# Autodesk Inventor assembly: ZMR250 Quadcopter Frame -Assembly
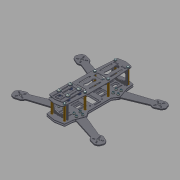
[picture p0: Inventor's stored thumbnail of the model, 180x180]
Saved by Autodesk Inventor 2011 SP2 (Build 150309200, 309)
## iProperties
Created: 2015-02-19
Part Number: ZMR250 Quadcopter Frame -Assembly
Document SubType Name: Assembly
Designer: Greg Pavlik
Author: Greg Pavlik
## Documents named in this file (15)
- C:\Users\Greg\Desktop\ZMR250 Quadcopter Frame\ZMR250 Quadcopter Frame -Assembly.iam
- C:\Users\Greg\Desktop\ZMR250 Quadcopter Frame\Bottom Plate.ipt
- C:\Users\Greg\Desktop\ZMR250 Quadcopter Frame\Arm.ipt
- C:\Users\Greg\Desktop\ZMR250 Quadcopter Frame\Spacer.ipt
- C:\Users\Greg\Desktop\ZMR250 Quadcopter Frame\Top Plate.ipt
- C:\Users\Greg\Desktop\ZMR250 Quadcopter Frame\Damper.ipt
- C:\Users\Greg\Desktop\ZMR250 Quadcopter Frame\Camera Plate.ipt
- C:\Users\Greg\Desktop\ZMR250 Quadcopter Frame\FPV Plate.ipt
- C:\Users\Greg\Desktop\ZMR250 Quadcopter Frame\Lock Washer.ipt
- C:\Users\Greg\Desktop\ZMR250 Quadcopter Frame\Hex Socket Screw.ipt
- C:\Users\Greg\Desktop\ZMR250 Quadcopter Frame\Hex Nut with Washer Face.ipt
- C:\Users\Greg\Desktop\ZMR250 Quadcopter Frame\Hex Head Cap Screw.ipt
- C:\Users\Greg\Desktop\ZMR250 Quadcopter Frame\Lock Washer -2.ipt
- C:\Users\Greg\Desktop\ZMR250 Quadcopter Frame\Round Head Machine Screw.ipt
- C:\Users\Greg\Desktop\ZMR250 Quadcopter Frame\Hex Jam Nut with Washer Face.ipt
## Components (134 placed, 14 different names)
1. Bottom Plate:1 — Flush:1, Flush:2, Mate:1, Mate:2, Mate:3, Mate:4, Mate:5, Mate:6, Mate:7, Mate:8, Mate:9, Mate:10, Mate:11, Mate:12, Mate:53, Mate:54, Insert:21, Insert:22, Insert:23, Insert:24, Insert:25, Insert:26, Insert:27, Insert:28, Insert:29, Insert:30, Insert:31, Insert:32, Insert:57, Insert:58, Insert:59, Insert:60, Insert:61, Insert:62, Insert:63, Insert:64
2. Bottom Plate:2 — Flush:1, Flush:2, Mate:13, Mate:14, Mate:15, Mate:16, Mate:17, Mate:18, Mate:19, Mate:20, Mate:21, Mate:22, Mate:23, Mate:24, Mate:25, Mate:26, Mate:27, Mate:28, Mate:29, Flush:7, Mate:41, Mate:42, Mate:43, Mate:44, Mate:45, Mate:46, Mate:47, Mate:48, Mate:49, Mate:50, Mate:51, Mate:52, Insert:9, Insert:10, Insert:11, Insert:12, Insert:13, Insert:14, Insert:15, Insert:16, Insert:17, Insert:18, Insert:19, Insert:20
3. Arm:1 — Mate:5, Mate:8, Mate:9
4. Arm:2 — Mate:6, Mate:7, Mate:12, Mate:13
5. Arm:3 — Mate:1, Mate:2, Mate:11
6. Arm:4 — Mate:3, Mate:4, Mate:10
7. Spacer:1 — Mate:15, Mate:27
8. Spacer:2 — Mate:20, Mate:29
9. Spacer:3 — Mate:21, Mate:28
10. Spacer:4 — Mate:14, Mate:22, Mate:31, Mate:32
11. Spacer:5 — Mate:16, Mate:26
12. Spacer:6 — Mate:17, Mate:23, Mate:30
13. Spacer:7 — Mate:18, Mate:24
14. Spacer:8 — Mate:19, Mate:25
15. Top Plate:1 — Mate:30, Mate:31, Mate:32, Mate:33, Mate:34, Mate:35, Mate:36, Mate:37, Insert:73, Insert:74, Insert:75, Insert:76, Insert:77, Insert:78, Insert:79, Insert:80
16. Damper:1 — Mate:33, Flush:5, Insert:92, Insert:94
17. Damper:2 — Mate:34, Flush:3, Flush:4, Mate:38, Mate:40, Insert:89, Insert:96
18. Damper:3 — Mate:35, Flush:4, Mate:37, Insert:91, Insert:95
19. Damper:4 — Mate:36, Flush:3, Flush:5, Mate:39, Insert:90, Insert:93
20. Camera Plate:1 — Mate:38, Mate:39, Mate:40
21. FPV Plate:1 — Flush:6, Flush:7, Mate:41, Mate:44
22. FPV Plate:2 — Flush:6, Mate:42, Mate:43
23. Lock Washer:1 — Flush:8, Mate:49, Insert:4
24. Lock Washer:2 — Flush:8, Flush:9, Mate:48, Insert:3
25. Lock Washer:3 — Flush:9, Flush:10, Mate:47, Insert:2
26. Lock Washer:4 — Flush:10, Mate:45, Mate:46, Insert:1
27. Lock Washer:5 — Flush:11, Mate:54, Insert:5
28. Lock Washer:6 — Mate:52, Flush:11, Flush:12, Insert:7
29. Lock Washer:7 — Mate:50, Flush:12, Flush:13, Mate:53, Insert:6
30. Lock Washer:8 — Mate:51, Flush:13, Insert:8
31. Lock Washer:9 — Insert:9, Insert:47
32. Lock Washer:10 — Insert:10, Insert:45
33. Lock Washer:11 — Insert:11, Insert:46
34. Lock Washer:12 — Insert:12, Insert:48
35. Lock Washer:13 — Insert:26, Insert:38
36. Lock Washer:14 — Insert:27, Insert:37
37. Lock Washer:15 — Insert:28, Insert:39
38. Lock Washer:16 — Insert:29, Insert:41
39. Lock Washer:17 — Insert:17, Insert:54
40. Lock Washer:18 — Insert:20, Insert:55
41. Lock Washer:19 — Insert:19, Insert:53
42. Lock Washer:20 — Insert:18, Insert:56
43. Lock Washer:21 — Insert:23, Insert:34
44. Lock Washer:22 — Insert:24, Insert:36
45. Lock Washer:23 — Insert:21, Insert:33
46. Lock Washer:24 — Insert:22, Insert:35
47. Lock Washer:25 — Insert:13, Insert:49
48. Lock Washer:26 — Insert:14, Insert:50
49. Lock Washer:27 — Insert:15, Insert:52
50. Lock Washer:28 — Insert:30, Insert:42
51. Lock Washer:29 — Insert:16, Insert:51
52. Lock Washer:30 — Insert:25, Insert:40
53. Lock Washer:31 — Insert:31, Insert:43
54. Lock Washer:32 — Insert:32, Insert:44
55. Hex Socket Screw:4 — Insert:4
56. Hex Nut with Washer Face:1 — Insert:8
57. Hex Nut with Washer Face:2 — Insert:7
58. Hex Nut with Washer Face:3 — Insert:5
59. Hex Nut with Washer Face:4 — Insert:6
60. Hex Nut with Washer Face:5 — Insert:41
61. Hex Nut with Washer Face:6 — Insert:42
62. Hex Nut with Washer Face:7 — Insert:43
63. Hex Nut with Washer Face:8 — Insert:44
64. Hex Nut with Washer Face:9 — Insert:37
65. Hex Nut with Washer Face:10 — Insert:38
66. Hex Nut with Washer Face:11 — Insert:39
67. Hex Nut with Washer Face:12 — Insert:40
68. Hex Nut with Washer Face:13 — Insert:36
69. Hex Nut with Washer Face:14 — Insert:35
70. Hex Nut with Washer Face:15 — Insert:34
71. Hex Nut with Washer Face:16 — Insert:33
72. Hex Socket Screw:1 — Insert:1
73. Hex Socket Screw:2 — Insert:2
74. Hex Socket Screw:3 — Insert:3
75. Hex Socket Screw:5 — Insert:49
76. Hex Socket Screw:6 — Insert:50
77. Hex Socket Screw:7 — Insert:51
78. Hex Socket Screw:8 — Insert:52
79. Hex Socket Screw:9 — Insert:53
80. Hex Socket Screw:10 — Insert:54
81. Hex Socket Screw:11 — Insert:55
82. Hex Socket Screw:12 — Insert:56
83. Hex Socket Screw:13 — Insert:45
84. Hex Socket Screw:14 — Insert:46
85. Hex Socket Screw:15 — Insert:47
86. Hex Socket Screw:16 — Insert:48
87. Lock Washer:33 — Insert:60, Insert:66
88. Lock Washer:34 — Insert:59, Insert:65
89. Lock Washer:35 — Insert:61, Insert:67
90. Lock Washer:36 — Insert:62, Insert:68
91. Lock Washer:37 — Insert:63, Insert:69
92. Lock Washer:38 — Insert:58, Insert:71
93. Lock Washer:39 — Insert:57, Insert:72
94. Lock Washer:40 — Insert:64, Insert:70
95. Hex Nut with Washer Face:17 — Insert:71
96. Hex Nut with Washer Face:18 — Insert:72
97. Hex Nut with Washer Face:19 — Insert:70
98. Hex Nut with Washer Face:20 — Insert:69
99. Hex Nut with Washer Face:21 — Insert:68
100. Hex Nut with Washer Face:22 — Insert:67
101. Hex Nut with Washer Face:23 — Insert:65
102. Hex Nut with Washer Face:24 — Insert:66
103. Lock Washer:41 — Insert:77, Insert:86
104. Lock Washer:42 — Insert:76, Insert:83
105. Lock Washer:43 — Insert:78, Insert:82
106. Lock Washer:44 — Insert:79, Insert:81
107. Lock Washer:45 — Insert:80, Insert:85
108. Lock Washer:46 — Insert:75, Insert:87
109. Lock Washer:47 — Insert:74, Insert:88
110. Lock Washer:48 — Insert:73, Insert:84
111. Hex Head Cap Screw:1 — Insert:81
112. Hex Head Cap Screw:2 — Insert:82
113. Hex Head Cap Screw:3 — Insert:83
114. Hex Head Cap Screw:4 — Insert:84
115. Hex Head Cap Screw:5 — Insert:85
116. Hex Head Cap Screw:6 — Insert:86
117. Hex Head Cap Screw:7 — Insert:87
118. Hex Head Cap Screw:8 — Insert:88
119. Lock Washer -2:1 — Insert:92, Insert:98
120. Lock Washer -2:2 — Insert:96, Insert:104
121. Lock Washer -2:3 — Insert:90, Insert:97
122. Lock Washer -2:4 — Insert:93, Insert:101
123. Lock Washer -2:5 — Insert:89, Insert:100
124. Lock Washer -2:6 — Insert:91, Insert:99
125. Lock Washer -2:7 — Insert:94, Insert:102
126. Lock Washer -2:8 — Insert:95, Insert:103
127. Round Head Machine Screw:1 — Insert:97
128. Round Head Machine Screw:2 — Insert:98
129. Round Head Machine Screw:3 — Insert:99
130. Round Head Machine Screw:4 — Insert:100
131. Hex Jam Nut with Washer Face:1 — Insert:101
132. Hex Jam Nut with Washer Face:2 — Insert:102
133. Hex Jam Nut with Washer Face:3 — Insert:104
134. Hex Jam Nut with Washer Face:4 — Insert:103
## Relationships (171: Insert 104, Mate 54, Flush 13)
- Flush:1: Bottom Plate:1 ↔ Bottom Plate:2
- Flush:2: Bottom Plate:1 ↔ Bottom Plate:2
- Mate:1: Bottom Plate:1 ↔ Arm:3
- Mate:2: Bottom Plate:1 ↔ Arm:3
- Mate:3: Bottom Plate:1 ↔ Arm:4
- Mate:4: Bottom Plate:1 ↔ Arm:4
- Mate:5: Bottom Plate:1 ↔ Arm:1
- Mate:6: Bottom Plate:1 ↔ Arm:2
- Mate:7: Bottom Plate:1 ↔ Arm:2
- Mate:8: Bottom Plate:1 ↔ Arm:1
- Mate:9: Bottom Plate:1 ↔ Arm:1
- Mate:10: Bottom Plate:1 ↔ Arm:4
- Mate:11: Bottom Plate:1 ↔ Arm:3
- Mate:12: Bottom Plate:1 ↔ Arm:2
- Mate:13: Bottom Plate:2 ↔ Arm:2
- Mate:14: Bottom Plate:2 ↔ Spacer:4
- Mate:15: Bottom Plate:2 ↔ Spacer:1
- Mate:16: Bottom Plate:2 ↔ Spacer:5
- Mate:17: Bottom Plate:2 ↔ Spacer:6
- Mate:18: Bottom Plate:2 ↔ Spacer:7
- Mate:19: Bottom Plate:2 ↔ Spacer:8
- Mate:20: Bottom Plate:2 ↔ Spacer:2
- Mate:21: Bottom Plate:2 ↔ Spacer:3
- Mate:22: Bottom Plate:2 ↔ Spacer:4
- Mate:23: Bottom Plate:2 ↔ Spacer:6
- Mate:24: Bottom Plate:2 ↔ Spacer:7
- Mate:25: Bottom Plate:2 ↔ Spacer:8
- Mate:26: Bottom Plate:2 ↔ Spacer:5
- Mate:27: Bottom Plate:2 ↔ Spacer:1
- Mate:28: Bottom Plate:2 ↔ Spacer:3
- Mate:29: Bottom Plate:2 ↔ Spacer:2
- Mate:30: Spacer:6 ↔ Top Plate:1
- Mate:31: Spacer:4 ↔ Top Plate:1
- Mate:32: Spacer:4 ↔ Top Plate:1
- Mate:33: Top Plate:1 ↔ Damper:1
- Mate:34: Top Plate:1 ↔ Damper:2
- Mate:35: Top Plate:1 ↔ Damper:3
- Mate:36: Top Plate:1 ↔ Damper:4
- Flush:3: Damper:2 ↔ Damper:4
- Flush:4: Damper:2 ↔ Damper:3
- Flush:5: Damper:1 ↔ Damper:4
- Mate:37: Top Plate:1 ↔ Damper:3
- Mate:38: Damper:2 ↔ Camera Plate:1
- Mate:39: Damper:4 ↔ Camera Plate:1
- Mate:40: Damper:2 ↔ Camera Plate:1
- Flush:6: FPV Plate:1 ↔ FPV Plate:2
- Flush:7: Bottom Plate:2 ↔ FPV Plate:1
- Mate:41: Bottom Plate:2 ↔ FPV Plate:1
- Mate:42: Bottom Plate:2 ↔ FPV Plate:2
- Mate:43: Bottom Plate:2 ↔ FPV Plate:2
- Mate:44: Bottom Plate:2 ↔ FPV Plate:1
- Flush:8: Lock Washer:1 ↔ Lock Washer:2
- Flush:9: Lock Washer:2 ↔ Lock Washer:3
- Flush:10: Lock Washer:3 ↔ Lock Washer:4
- Mate:45: Bottom Plate:2 ↔ Lock Washer:4
- Mate:46: Bottom Plate:2 ↔ Lock Washer:4
- Mate:47: Bottom Plate:2 ↔ Lock Washer:3
- Mate:48: Bottom Plate:2 ↔ Lock Washer:2
- Mate:49: Bottom Plate:2 ↔ Lock Washer:1
- Mate:50: Bottom Plate:2 ↔ Lock Washer:7
- Mate:51: Bottom Plate:2 ↔ Lock Washer:8
- Mate:52: Bottom Plate:2 ↔ Lock Washer:6
- Flush:11: Lock Washer:5 ↔ Lock Washer:6
- Flush:12: Lock Washer:6 ↔ Lock Washer:7
- Flush:13: Lock Washer:7 ↔ Lock Washer:8
- Mate:53: Bottom Plate:1 ↔ Lock Washer:7
- Mate:54: Bottom Plate:1 ↔ Lock Washer:5
- Insert:1: Lock Washer:4 ↔ Hex Socket Screw:1
- Insert:2: Lock Washer:3 ↔ Hex Socket Screw:2
- Insert:3: Lock Washer:2 ↔ Hex Socket Screw:3
- Insert:4: Lock Washer:1 ↔ Hex Socket Screw:4
- Insert:5: Lock Washer:5 ↔ Hex Nut with Washer Face:3
- Insert:6: Lock Washer:7 ↔ Hex Nut with Washer Face:4
- Insert:7: Lock Washer:6 ↔ Hex Nut with Washer Face:2
- Insert:8: Lock Washer:8 ↔ Hex Nut with Washer Face:1
- Insert:9: Bottom Plate:2 ↔ Lock Washer:9
- Insert:10: Bottom Plate:2 ↔ Lock Washer:10
- Insert:11: Bottom Plate:2 ↔ Lock Washer:11
- Insert:12: Bottom Plate:2 ↔ Lock Washer:12
- Insert:13: Bottom Plate:2 ↔ Lock Washer:25
- Insert:14: Bottom Plate:2 ↔ Lock Washer:26
- Insert:15: Bottom Plate:2 ↔ Lock Washer:27
- Insert:16: Bottom Plate:2 ↔ Lock Washer:29
- Insert:17: Bottom Plate:2 ↔ Lock Washer:17
- Insert:18: Bottom Plate:2 ↔ Lock Washer:20
- Insert:19: Bottom Plate:2 ↔ Lock Washer:19
- Insert:20: Bottom Plate:2 ↔ Lock Washer:18
- Insert:21: Bottom Plate:1 ↔ Lock Washer:23
- Insert:22: Bottom Plate:1 ↔ Lock Washer:24
- Insert:23: Bottom Plate:1 ↔ Lock Washer:21
- Insert:24: Bottom Plate:1 ↔ Lock Washer:22
- Insert:25: Bottom Plate:1 ↔ Lock Washer:30
- Insert:26: Bottom Plate:1 ↔ Lock Washer:13
- Insert:27: Bottom Plate:1 ↔ Lock Washer:14
- Insert:28: Bottom Plate:1 ↔ Lock Washer:15
- Insert:29: Bottom Plate:1 ↔ Lock Washer:16
- Insert:30: Bottom Plate:1 ↔ Lock Washer:28
- Insert:31: Bottom Plate:1 ↔ Lock Washer:31
- Insert:32: Bottom Plate:1 ↔ Lock Washer:32
- Insert:33: Lock Washer:23 ↔ Hex Nut with Washer Face:16
- Insert:34: Lock Washer:21 ↔ Hex Nut with Washer Face:15
- Insert:35: Lock Washer:24 ↔ Hex Nut with Washer Face:14
- Insert:36: Lock Washer:22 ↔ Hex Nut with Washer Face:13
- Insert:37: Lock Washer:14 ↔ Hex Nut with Washer Face:9
- Insert:38: Lock Washer:13 ↔ Hex Nut with Washer Face:10
- Insert:39: Lock Washer:15 ↔ Hex Nut with Washer Face:11
- Insert:40: Lock Washer:30 ↔ Hex Nut with Washer Face:12
- Insert:41: Lock Washer:16 ↔ Hex Nut with Washer Face:5
- Insert:42: Lock Washer:28 ↔ Hex Nut with Washer Face:6
- Insert:43: Lock Washer:31 ↔ Hex Nut with Washer Face:7
- Insert:44: Lock Washer:32 ↔ Hex Nut with Washer Face:8
- Insert:45: Lock Washer:10 ↔ Hex Socket Screw:13
- Insert:46: Lock Washer:11 ↔ Hex Socket Screw:14
- Insert:47: Lock Washer:9 ↔ Hex Socket Screw:15
- Insert:48: Lock Washer:12 ↔ Hex Socket Screw:16
- Insert:49: Lock Washer:25 ↔ Hex Socket Screw:5
- Insert:50: Lock Washer:26 ↔ Hex Socket Screw:6
- Insert:51: Lock Washer:29 ↔ Hex Socket Screw:7
- Insert:52: Lock Washer:27 ↔ Hex Socket Screw:8
- Insert:53: Lock Washer:19 ↔ Hex Socket Screw:9
- Insert:54: Lock Washer:17 ↔ Hex Socket Screw:10
- Insert:55: Lock Washer:18 ↔ Hex Socket Screw:11
- Insert:56: Lock Washer:20 ↔ Hex Socket Screw:12
- Insert:57: Bottom Plate:1 ↔ Lock Washer:39
- Insert:58: Bottom Plate:1 ↔ Lock Washer:38
- Insert:59: Bottom Plate:1 ↔ Lock Washer:34
- Insert:60: Bottom Plate:1 ↔ Lock Washer:33
- Insert:61: Bottom Plate:1 ↔ Lock Washer:35
- Insert:62: Bottom Plate:1 ↔ Lock Washer:36
- Insert:63: Bottom Plate:1 ↔ Lock Washer:37
- Insert:64: Bottom Plate:1 ↔ Lock Washer:40
- Insert:65: Lock Washer:34 ↔ Hex Nut with Washer Face:23
- Insert:66: Lock Washer:33 ↔ Hex Nut with Washer Face:24
- Insert:67: Lock Washer:35 ↔ Hex Nut with Washer Face:22
- Insert:68: Lock Washer:36 ↔ Hex Nut with Washer Face:21
- Insert:69: Lock Washer:37 ↔ Hex Nut with Washer Face:20
- Insert:70: Lock Washer:40 ↔ Hex Nut with Washer Face:19
- Insert:71: Lock Washer:38 ↔ Hex Nut with Washer Face:17
- Insert:72: Lock Washer:39 ↔ Hex Nut with Washer Face:18
- Insert:73: Top Plate:1 ↔ Lock Washer:48
- Insert:74: Top Plate:1 ↔ Lock Washer:47
- Insert:75: Top Plate:1 ↔ Lock Washer:46
- Insert:76: Top Plate:1 ↔ Lock Washer:42
- Insert:77: Top Plate:1 ↔ Lock Washer:41
- Insert:78: Top Plate:1 ↔ Lock Washer:43
- Insert:79: Top Plate:1 ↔ Lock Washer:44
- Insert:80: Top Plate:1 ↔ Lock Washer:45
- Insert:81: Lock Washer:44 ↔ Hex Head Cap Screw:1
- Insert:82: Lock Washer:43 ↔ Hex Head Cap Screw:2
- Insert:83: Lock Washer:42 ↔ Hex Head Cap Screw:3
- Insert:84: Lock Washer:48 ↔ Hex Head Cap Screw:4
- Insert:85: Lock Washer:45 ↔ Hex Head Cap Screw:5
- Insert:86: Lock Washer:41 ↔ Hex Head Cap Screw:6
- Insert:87: Lock Washer:46 ↔ Hex Head Cap Screw:7
- Insert:88: Lock Washer:47 ↔ Hex Head Cap Screw:8
- Insert:89: Damper:2 ↔ Lock Washer -2:5
- Insert:90: Damper:4 ↔ Lock Washer -2:3
- Insert:91: Damper:3 ↔ Lock Washer -2:6
- Insert:92: Damper:1 ↔ Lock Washer -2:1
- Insert:93: Damper:4 ↔ Lock Washer -2:4
- Insert:94: Damper:1 ↔ Lock Washer -2:7
- Insert:95: Damper:3 ↔ Lock Washer -2:8
- Insert:96: Damper:2 ↔ Lock Washer -2:2
- Insert:97: Lock Washer -2:3 ↔ Round Head Machine Screw:1
- Insert:98: Lock Washer -2:1 ↔ Round Head Machine Screw:2
- Insert:99: Lock Washer -2:6 ↔ Round Head Machine Screw:3
- Insert:100: Lock Washer -2:5 ↔ Round Head Machine Screw:4
- Insert:101: Lock Washer -2:4 ↔ Hex Jam Nut with Washer Face:1
- Insert:102: Lock Washer -2:7 ↔ Hex Jam Nut with Washer Face:2
- Insert:103: Lock Washer -2:8 ↔ Hex Jam Nut with Washer Face:4
- Insert:104: Lock Washer -2:2 ↔ Hex Jam Nut with Washer Face:3
